# Autodesk Inventor assembly: AM14U4 Square
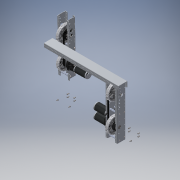
[picture p0: Inventor's stored thumbnail of the model, 180x180]
Saved by Autodesk Inventor 2017 (Build 210142000, 142)
## iProperties
Created: 2018-10-11
Part Number: AM14U4 Square
Material: 一般
Description: STEP AP214
Document SubType Name: Assembly
Designer: IJA
Sending System: SolidWorks 2018
Preprocessor: SwSTEP 2.0
Title: AM14U4 Square.STEP
Revision Number: ANY
## Documents named in this file (11)
- D:\Works\Robot2\AM14U4 Square.iam
- D:\Works\Robot2\AM14U4 Square Half.iam
- D:\Works\Robot2\am-xxxx AM14U4 Outside Plate Square_DefaultSM-FLAT-PATTERN_MIR.ipt
- D:\Works\Robot2\am-xxxx AM14U4 Outside Plate Square_DefaultSM-FLAT-PATTERN.ipt
- D:\Works\Robot2\AM14U4 Square Half2.iam
- D:\Works\Robot2\am-xxxx AM14U4 Inside Plate Square.ipt
- D:\Works\Robot2\6 HiGrip with bearings, pulleys and spacers.iam
- D:\Works\Robot2\375-16 x 4.25 Hex Bolt_HFBOLT 0.375-16x2.5x1-C.ipt
- D:\Works\Robot2\3-8-16 NyLock Nut - Mcm 95615A140_95615A140.ipt
- D:\Works\Robot2\655-5M-15 v2.ipt
- D:\Works\Robot2\am-xxxx AM14U4 End Plate Square2.ipt
## Components (11 placed, 11 different names)
1. AM14U4 Square Half_1 [sub-assembly] — 角度:8
2. 655-5M-15 v2_9 — 貼合:6
3. 6 HiGrip with bearings, pulleys and spacers_4 [sub-assembly] — 貼合:3
4. 375-16 x 4.25 Hex Bolt_HFBOLT 0.375-16x2.5x1-C_11 — 貼合:4
5. 3-8-16 NyLock Nut - Mcm 95615A140_95615A140_13
6. AM14U4 Square Half_2 [sub-assembly]
7. am-xxxx AM14U4 Outside Plate Square_DefaultSM-FLAT-PATTERN_83
8. am-xxxx AM14U4 Inside Plate Square_84 — 角度:4, 貼合:2, 貼合:3, 貼合:4, 角度:8
9. am-xxxx AM14U4 Outside Plate Square_DefaultSM-FLAT-PATTERN_MIR:1 — 角度:4, 貼合:7
10. AM14U4 Square Half2:1 [sub-assembly] — 貼合:2, 貼合:6
11. am-xxxx AM14U4 End Plate Square2:1 — 貼合:7
## Relationships (10: Angle 5, Mate 5)
- 角度:4 [Angle] (0 deg): am-xxxx AM14U4 Inside Plate Square_84 ↔ am-xxxx AM14U4 Outside Plate Square_DefaultSM-FLAT-PATTERN_MIR:1
- 貼合:2 [Mate]: am-xxxx AM14U4 Inside Plate Square_84 ↔ AM14U4 Square Half2:1
- [Angle] (0 deg): 6 HiGrip with bearings, pulleys and spacers_4 ↔ AM14U4 Square Half2:1
- [Angle] (0 deg): 6 HiGrip with bearings, pulleys and spacers_4 ↔ 375-16 x 4.25 Hex Bolt_HFBOLT 0.375-16x2.5x1-C_11
- 貼合:3 [Mate]: 6 HiGrip with bearings, pulleys and spacers_4 ↔ am-xxxx AM14U4 Inside Plate Square_84
- [Angle] (0 deg): 375-16 x 4.25 Hex Bolt_HFBOLT 0.375-16x2.5x1-C_11 ↔ 3-8-16 NyLock Nut - Mcm 95615A140_95615A140_13
- 貼合:4 [Mate]: 375-16 x 4.25 Hex Bolt_HFBOLT 0.375-16x2.5x1-C_11 ↔ am-xxxx AM14U4 Inside Plate Square_84
- 貼合:6 [Mate]: 655-5M-15 v2_9 ↔ AM14U4 Square Half2:1
- 角度:8 [Angle] (0 deg): AM14U4 Square Half_1 ↔ am-xxxx AM14U4 Inside Plate Square_84
- 貼合:7 [Mate]: am-xxxx AM14U4 Outside Plate Square_DefaultSM-FLAT-PATTERN_MIR:1 ↔ am-xxxx AM14U4 End Plate Square2:1
